# Autodesk Inventor assembly: Assembly_V2
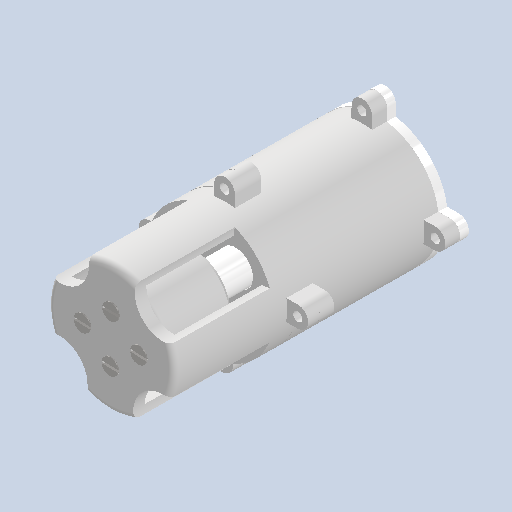
[picture p0: Inventor's stored thumbnail of the model, 512x512]
Saved by Autodesk Inventor 2025.2 (Build 292293000, 293)
## iProperties
Created: 2023-12-14
Part Number: Assembly_V2
Document SubType Name: Assembly
Designer: mirun
Author: mirun
## Documents named in this file (10)
- C:\Users\mirewn\Documents\GitHub\Electric-Screwdriver\GearBox\Assembly.iam
- C:\Users\mirewn\Documents\GitHub\Electric-Screwdriver\GearBox\ring.ipt
- C:\Users\mirewn\Documents\GitHub\Electric-Screwdriver\GearBox\motor_adaptor.ipt
- C:\Users\mirewn\Documents\GitHub\Electric-Screwdriver\GearBox\plnetgear.ipt
- C:\Users\mirewn\Documents\GitHub\Electric-Screwdriver\GearBox\carrier.ipt
- C:\Users\mirewn\Documents\GitHub\Electric-Screwdriver\GearBox\ax.ipt
- C:\Users\mirewn\Documents\GitHub\Electric-Screwdriver\GearBox\lid.ipt
- C:\Users\mirewn\OneDrive - Universitatea Politehnica Bucuresti\AA- Projects\Surubelnita\Capac_MOTOR.ipt
- C:\Users\mirewn\OneDrive - Universitatea Politehnica Bucuresti\AA- Projects\Surubelnita\motor.ipt
- C:\Users\mirewn\Documents\Inventor\Content Center Files\R2025\en-US\DIN 963\DIN 963 - M3 x 6.ipt
## Components (24 placed, 9 different names)
1. ring:1 — Mate:8, Mate:16, Mate:23, Mate:24, Flush:5, Mate:29, Mate:30, Mate:31, Mate:36
2. motor_adaptor:1 — Mate:8, Mate:15, Mate:26, Mate:27, Mate:28
3. carrier:1 — Mate:11, Mate:12, Mate:15, Mate:17, Mate:18, Mate:28
4. carrier:2 — Mate:13, Mate:14, Mate:18, Mate:21, Mate:22
5. ax:1 — Mate:19, Mate:20, Mate:22
6. lid:1 — Mate:23, Mate:24, Mate:31
7. motor:1 — Mate:26, Mate:27
8. Capac_MOTOR:1 — Flush:5, Mate:29, Mate:30, Mate:32, Mate:33, Mate:34, Mate:35, Mate:36
9. DIN 963 - replaced by DIN EN ISO 2009 M3 x 6:1 — Mate:32
10. DIN 963 - replaced by DIN EN ISO 2009 M3 x 6:2 — Mate:33
11. DIN 963 - replaced by DIN EN ISO 2009 M3 x 6:3 — Mate:34
12. DIN 963 - replaced by DIN EN ISO 2009 M3 x 6:4 — Mate:35
13. plnetgear:1 — Mate:11, Mate:12
14. plnetgear:2
15. plnetgear:3
16. plnetgear:4 — Mate:16
17. plnetgear:9 — Mate:13, Mate:14
18. plnetgear:10
19. plnetgear:11 — Mate:17
20. plnetgear:12
21. plnetgear:5 — Mate:19, Mate:20, Mate:21
22. plnetgear:6
23. plnetgear:7
24. plnetgear:8
## Component patterns: (4 elements, first: plnetgear:1), (4 elements, first: plnetgear:9), (4 elements, first: plnetgear:5)
## Relationships (27: Mate 26, Flush 1)
- Mate:8: ring:1 ↔ motor_adaptor:1
- Mate:11: carrier:1 ↔ plnetgear:1
- Mate:12: carrier:1 ↔ plnetgear:1
- Mate:13: carrier:2 ↔ plnetgear:9
- Mate:14: carrier:2 ↔ plnetgear:9
- Mate:15: motor_adaptor:1 ↔ carrier:1
- Mate:16: ring:1 ↔ plnetgear:4
- Mate:17: carrier:1 ↔ plnetgear:11
- Mate:18: carrier:1 ↔ carrier:2
- Mate:19: ax:1 ↔ plnetgear:5
- Mate:20: ax:1 ↔ plnetgear:5
- Mate:21: carrier:2 ↔ plnetgear:5
- Mate:22: carrier:2 ↔ ax:1
- Mate:23: ring:1 ↔ lid:1
- Mate:24: ring:1 ↔ lid:1
- Mate:26: motor_adaptor:1 ↔ motor:1
- Mate:27: motor_adaptor:1 ↔ motor:1
- Flush:5: ring:1 ↔ Capac_MOTOR:1
- Mate:28: motor_adaptor:1 ↔ carrier:1
- Mate:29: ring:1 ↔ Capac_MOTOR:1
- Mate:30: ring:1 ↔ Capac_MOTOR:1
- Mate:31: ring:1 ↔ lid:1
- Mate:32: Capac_MOTOR:1 ↔ DIN 963 - replaced by DIN EN ISO 2009 M3 x 6:1
- Mate:33: Capac_MOTOR:1 ↔ DIN 963 - replaced by DIN EN ISO 2009 M3 x 6:2
- Mate:34: Capac_MOTOR:1 ↔ DIN 963 - replaced by DIN EN ISO 2009 M3 x 6:3
- Mate:35: Capac_MOTOR:1 ↔ DIN 963 - replaced by DIN EN ISO 2009 M3 x 6:4
- Mate:36: ring:1 ↔ Capac_MOTOR:1
